# Autodesk Inventor assembly: platform_0606_fig2_ratio12
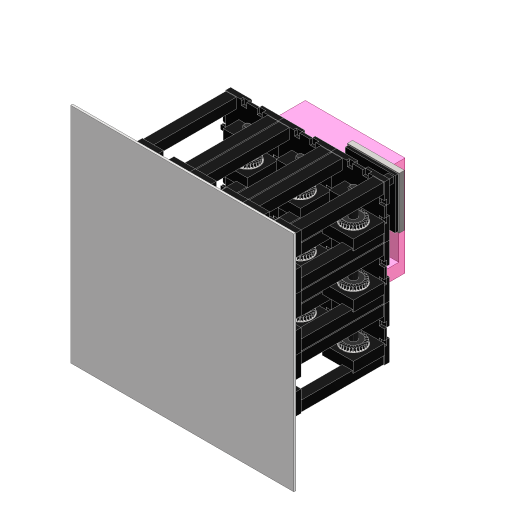
[picture p0: Inventor's stored thumbnail of the model, 512x512]
Saved by Autodesk Inventor 2024 (Build 280153000, 153)
## iProperties
Created: 2024-06-06
Part Number: platform_0606_fig2_ratio12
Document SubType Name: Assembly
Designer: admin
Author: admin
## Documents named in this file (9)
- C:\Users\admin\OneDrive\文件\碩士研究\prototype\plane_unit_0606\platform_0606_fig2_ratio12.iam
- C:\Users\admin\OneDrive\文件\碩士研究\prototype\plane_unit_0606\one_way_bearing.ipt
- C:\Users\admin\OneDrive\文件\碩士研究\prototype\plane_unit_0606\printer_base_plane.ipt
- C:\Users\admin\OneDrive\文件\碩士研究\prototype\plane_unit_0606\rod_1221.ipt
- C:\Users\admin\OneDrive\文件\碩士研究\prototype\plane_unit_0606\iron_plate.ipt
- C:\Users\admin\OneDrive\文件\碩士研究\prototype\plane_unit_0606\plane_unit_1121.ipt
- C:\Users\admin\OneDrive\文件\碩士研究\prototype\plane_unit_0606\gear_pin_1222_.ipt
- C:\Users\admin\OneDrive\文件\碩士研究\prototype\plane_unit_0606\bridge_rect_final_12.ipt
- C:\Users\admin\OneDrive\文件\碩士研究\prototype\plane_unit_0606\trimmed_block_12.ipt
## Components (32 placed, 8 different names)
1. printer_base_plane:1 — 貼合:1, 齊平:1, 齊平:2, 齊平:4, 齊平:5, 25, 貼合:12
2. rod_1221:1 — 貼合:7, 貼合:8, 貼合:9, 貼合:10, 貼合:11
3. iron_plate:1 — 貼合:9, 貼合:10, 貼合:11, 齊平:4
4. bridge_rect_final_12:1 — 齊平:5, 25, 貼合:12, 貼合:13, 齊平:7, 貼合:14
5. trimmed_block_12:1 — 貼合:13, 齊平:7, 貼合:14
6. one_way_bearing:1 — 貼合:2, 齊平:3, 貼合:3, 貼合:4
7. plane_unit_1121:1 — 貼合:1, 齊平:1, 齊平:2, 貼合:2, 齊平:3, 貼合:7, 貼合:8
8. gear_pin_1222_:1 — 貼合:3, 貼合:4
9. one_way_bearing:2
10. plane_unit_1121:2
11. gear_pin_1222_:2
12. one_way_bearing:3
13. plane_unit_1121:3
14. gear_pin_1222_:3
15. one_way_bearing:4
16. plane_unit_1121:4
17. gear_pin_1222_:4
18. one_way_bearing:5
19. plane_unit_1121:5
20. gear_pin_1222_:5
21. one_way_bearing:6
22. plane_unit_1121:6
23. gear_pin_1222_:6
24. one_way_bearing:7
25. plane_unit_1121:7
26. gear_pin_1222_:7
27. one_way_bearing:8
28. plane_unit_1121:8
29. gear_pin_1222_:8
30. one_way_bearing:9
31. plane_unit_1121:9
32. gear_pin_1222_:9
## Component patterns: (9 elements, first: one_way_bearing:1 + plane_unit_1121:1 + gear_pin_1222_:1)
## Relationships (19: Mate 12, Flush 7)
- 貼合:1 [Mate]: printer_base_plane:1 ↔ plane_unit_1121:1
- 齊平:1 [Flush] (5 mm): printer_base_plane:1 ↔ plane_unit_1121:1
- 齊平:2 [Flush] (5 mm): printer_base_plane:1 ↔ plane_unit_1121:1
- 貼合:2 [Mate]: one_way_bearing:1 ↔ plane_unit_1121:1
- 齊平:3 [Flush]: one_way_bearing:1 ↔ plane_unit_1121:1
- 貼合:3 [Mate]: one_way_bearing:1 ↔ gear_pin_1222_:1
- 貼合:4 [Mate]: one_way_bearing:1 ↔ gear_pin_1222_:1
- 貼合:7 [Mate] (0.2 mm): rod_1221:1 ↔ plane_unit_1121:1
- 貼合:8 [Mate] (0.2 mm): rod_1221:1 ↔ plane_unit_1121:1
- 貼合:9 [Mate]: rod_1221:1 ↔ iron_plate:1
- 貼合:10 [Mate]: rod_1221:1 ↔ iron_plate:1
- 貼合:11 [Mate]: rod_1221:1 ↔ iron_plate:1
- 齊平:4 [Flush] (-110 mm): printer_base_plane:1 ↔ iron_plate:1
- 齊平:5 [Flush] (35 mm): printer_base_plane:1 ↔ bridge_rect_final_12:1
- 25 [Flush] (25 mm): printer_base_plane:1 ↔ bridge_rect_final_12:1
- 貼合:12 [Mate] (110 mm): printer_base_plane:1 ↔ bridge_rect_final_12:1
- 貼合:13 [Mate]: bridge_rect_final_12:1 ↔ trimmed_block_12:1
- 齊平:7 [Flush]: bridge_rect_final_12:1 ↔ trimmed_block_12:1
- 貼合:14 [Mate]: bridge_rect_final_12:1 ↔ trimmed_block_12:1
